# Autodesk Inventor assembly: PCBPT_V3_V2
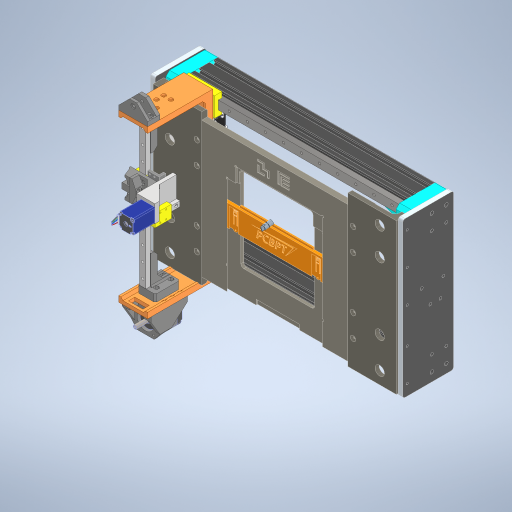
[picture p0: Inventor's stored thumbnail of the model, 512x512]
Saved by Autodesk Inventor 2024.1 (Build 281209000, 209)
## iProperties
Created: 2023-09-27
Part Number: PCBPT_V3_V2
Document SubType Name: Assembly
Designer: l1534
Author: l1534
## Documents named in this file (29)
- C:\DATA\Documents\Lab\github\PCBPT\PCBPT_V3\Mechanical\Mechanical_2\PCBPT_V3_V2.iam
- C:\DATA\Documents\Lab\github\PCBPT\PCBPT_V3\Mechanical\Mechanical_2\Nema 17 Stepper Motor - 40mm - 1.8deg, 61oz-in v1 (2).ipt
- C:\DATA\Documents\Lab\github\PCBPT\PCBPT_V3\Mechanical\Mechanical_2\Part 1 (1).ipt
- C:\DATA\Documents\Lab\github\PCBPT\PCBPT_V3\Mechanical\Mechanical_2\Part 1 (2).ipt
- C:\DATA\Documents\Lab\github\PCBPT\PCBPT_V3\Mechanical\Mechanical_2\Part 1 (3).ipt
- C:\DATA\Documents\Lab\github\PCBPT\PCBPT_V3\Mechanical\Mechanical_2\Part 1 (6).ipt
- C:\DATA\Documents\Lab\github\PCBPT\PCBPT_V3\Mechanical\Mechanical_2\Part 1 (21).ipt
- C:\DATA\Documents\Lab\github\PCBPT\PCBPT_V3\Mechanical\Mechanical_2\Part 1 (22).ipt
- C:\DATA\Documents\Lab\github\PCBPT\PCBPT_V3\Mechanical\Mechanical_2\Part 1 (23).ipt
- C:\DATA\Documents\Lab\github\PCBPT\PCBPT_V3\Mechanical\Mechanical_2\Part Studio 1 - Part 1.ipt
- C:\DATA\Documents\Lab\github\PCBPT\PCBPT_V3\Mechanical\Mechanical_2\wall_conn_2 v8 (2).ipt
- C:\DATA\Documents\Lab\github\PCBPT\PCBPT_V3\Mechanical\Mechanical_2\Wall_connector v11 (2).ipt
- C:\DATA\Documents\Lab\github\PCBPT\PCBPT_V3\Mechanical\Mechanical_2\MGN12H_block.ipt
- C:\DATA\Documents\Lab\github\PCBPT\PCBPT_V3\Mechanical\Mechanical_2\MGN12H_rail.ipt
- C:\DATA\Documents\Lab\github\PCBPT\PCBPT_V3\Mechanical\Mechanical_2\MGN9C_block.ipt
- C:\DATA\Documents\Lab\github\PCBPT\PCBPT_V3\Mechanical\Mechanical_2\MGN9x200mm_rail.ipt
- C:\DATA\Documents\Lab\github\PCBPT\PCBPT_V3\Mechanical\6mm 3v laser diode (1)\6mm 3v laser diode (1).ipt
- C:\DATA\Documents\Lab\github\PCBPT\PCBPT_V3\Mechanical\Part 1 (33)\Part 1 (33).ipt
- C:\DATA\Documents\Lab\github\PCBPT\PCBPT_V3\Mechanical\Mechanical_2\Part 1 (41)\Part 1 (41).ipt
- C:\DATA\Documents\Lab\github\PCBPT\PCBPT_V3\Mechanical\Mechanical_2\Part 1 (83)\Part 1 (83).ipt
- C:\DATA\Documents\Lab\github\PCBPT\PCBPT_V3\Mechanical\Mechanical_2\Part 1 (7)\Part 1 (7).ipt
- C:\DATA\Documents\Lab\github\PCBPT\PCBPT_V3\Mechanical\Mechanical_2\SY20STH30-0604A (2)\SY20STH30-0604A (2).ipt
- C:\DATA\Documents\Lab\github\PCBPT\PCBPT_V3\Mechanical\Mechanical_2\Z_motor_holder.ipt
- C:\DATA\Documents\Lab\github\PCBPT\PCBPT_V3\Mechanical\Mechanical_2\MGN7c_50mm_rail.ipt
- C:\DATA\Documents\Lab\github\PCBPT\PCBPT_V3\Mechanical\Mechanical_2\MGN7C_slider.ipt
- C:\DATA\Documents\Lab\github\PCBPT\PCBPT_V3\Mechanical\Mechanical_2\platform - Part 1\platform - Part 1.ipt
- C:\DATA\Documents\Lab\github\PCBPT\PCBPT_V3\Mechanical\Mechanical_2\PCB_clip - Part 1\PCB_clip - Part 1.ipt
- C:\DATA\Documents\Lab\github\PCBPT\PCBPT_V3\Mechanical\Mechanical_2\platform_holder_L - Part 1\platform_holder_L - Part 1.ipt
- C:\DATA\Documents\Lab\github\PCBPT\PCBPT_V3\Mechanical\Mechanical_2\platform_holder_R - Part 1\platform_holder_R - Part 1.ipt
## Components (36 placed, 28 different names)
1. Nema 17 Stepper Motor - 40mm - 1.8deg, 61oz-in v1 (2):1 — Rigid:11
2. Part 1 (1):1 — Rigid:14, Rigid:15, Rigid:16, Rigid:17, Rigid:18, Rigid:25
3. Part 1 (2):1 — Rigid:9, Rigid:11
4. Part 1 (23):1 — Rigid:6, Rigid:7, Mate:6
5. Part Studio 1 - Part 1:1 — Rigid:3, Rigid:4, Rigid:8, Rigid:30
6. wall_conn_2 v8 (2):1 — Rigid:4, Mate:4, Flush:1
7. Wall_connector v11 (2):1 — Rigid:3, Rigid:7, Mate:5
8. Nema 17 Stepper Motor - 40mm - 1.8deg, 61oz-in v1 (2):2 — Rigid:10
9. Part 1 (2):2 — Rigid:8, Rigid:10
10. Part 1 (3):2 — Rigid:16
11. Part 1 (6):2 — Rigid:17, Rigid:20
12. Part 1 (21):2 — Rigid:19
13. Part 1 (22):2 — Rigid:18, Rigid:19
14. Part 1 (23):2 — Rigid:5, Mate:3
15. Part Studio 1 - Part 1:2 — Rigid:1, Rigid:2, Rigid:9, Rigid:29
16. wall_conn_2 v8 (2):2 — Rigid:2, Rigid:6
17. Wall_connector v11 (2):2 — Rigid:1, Rigid:5
18. MGN12H_rail:1 — Mate:2, Mate:3, Mate:4, Flush:1
19. MGN12H_rail:2 — Mate:1, Mate:5, Mate:6
20. MGN12H_block:3 — Rigid:14, Mate:2
21. MGN12H_block:4 — Rigid:15, Mate:1
22. MGN9C_block:1 — Mate:7, Mate:8, Rigid:24
23. MGN9x200mm_rail:1 — Rigid:20, Mate:7, Mate:8
24. 6mm 3v laser diode (1):1
25. Part 1 (33):1 — Rigid:22, Rigid:23, Rigid:24, Rigid:28
26. Part 1 (41):1 — Rigid:22
27. Part 1 (83):1 — Rigid:23
28. Part 1 (7):1 — Rigid:25
29. SY20STH30-0604A (2):1 — Rigid:27
30. Z_motor_holder:1 — Rigid:26, Rigid:27, Rigid:28
31. MGN7c_50mm_rail:1 — Rigid:26, Mate:9, Mate:10
32. MGN7C_slider:1 — Mate:9, Mate:10
33. platform - Part 1:1 — Rigid:31, Mate:11, Mate:12
34. PCB_clip - Part 1:1 — Mate:11, Mate:12
35. platform_holder_L - Part 1:1 — Rigid:29
36. platform_holder_R - Part 1:1 — Rigid:30, Rigid:31
## Relationships (41: WeldJoint 28, Mate 12, Flush 1)
- Rigid:1 [WeldJoint]: Part Studio 1 - Part 1:2 ↔ Wall_connector v11 (2):2
- Rigid:2 [WeldJoint]: Part Studio 1 - Part 1:2 ↔ wall_conn_2 v8 (2):2
- Rigid:3 [WeldJoint]: Part Studio 1 - Part 1:1 ↔ Wall_connector v11 (2):1
- Rigid:4 [WeldJoint]: Part Studio 1 - Part 1:1 ↔ wall_conn_2 v8 (2):1
- Rigid:5 [WeldJoint]: Part 1 (23):2 ↔ Wall_connector v11 (2):2
- Rigid:6 [WeldJoint]: Part 1 (23):1 ↔ wall_conn_2 v8 (2):2
- Rigid:7 [WeldJoint]: Part 1 (23):1 ↔ Wall_connector v11 (2):1
- Rigid:8 [WeldJoint]: Part Studio 1 - Part 1:1 ↔ Part 1 (2):2
- Rigid:9 [WeldJoint]: Part 1 (2):1 ↔ Part Studio 1 - Part 1:2
- Rigid:10 [WeldJoint]: Nema 17 Stepper Motor - 40mm - 1.8deg, 61oz-in v1 (2):2 ↔ Part 1 (2):2
- Rigid:11 [WeldJoint]: Nema 17 Stepper Motor - 40mm - 1.8deg, 61oz-in v1 (2):1 ↔ Part 1 (2):1
- Rigid:14 [WeldJoint]: Part 1 (1):1 ↔ MGN12H_block:3
- Rigid:15 [WeldJoint]: Part 1 (1):1 ↔ MGN12H_block:4
- Rigid:16 [WeldJoint]: Part 1 (1):1 ↔ Part 1 (3):2
- Rigid:17 [WeldJoint]: Part 1 (1):1 ↔ Part 1 (6):2
- Rigid:18 [WeldJoint]: Part 1 (1):1 ↔ Part 1 (22):2
- Rigid:19 [WeldJoint]: Part 1 (21):2 ↔ Part 1 (22):2
- Mate:1: MGN12H_rail:2 ↔ MGN12H_block:4
- Mate:2: MGN12H_rail:1 ↔ MGN12H_block:3
- Mate:3: Part 1 (23):2 ↔ MGN12H_rail:1
- Mate:4: wall_conn_2 v8 (2):1 ↔ MGN12H_rail:1
- Flush:1 (4 mm): wall_conn_2 v8 (2):1 ↔ MGN12H_rail:1
- Mate:5: Wall_connector v11 (2):1 ↔ MGN12H_rail:2
- Mate:6: Part 1 (23):1 ↔ MGN12H_rail:2
- Rigid:20 [WeldJoint]: Part 1 (6):2 ↔ MGN9x200mm_rail:1
- Mate:7: MGN9C_block:1 ↔ MGN9x200mm_rail:1
- Mate:8: MGN9C_block:1 ↔ MGN9x200mm_rail:1
- Rigid:22 [WeldJoint]: Part 1 (33):1 ↔ Part 1 (41):1
- Rigid:23 [WeldJoint]: Part 1 (33):1 ↔ Part 1 (83):1
- Rigid:24 [WeldJoint]: MGN9C_block:1 ↔ Part 1 (33):1
- Rigid:25 [WeldJoint]: Part 1 (1):1 ↔ Part 1 (7):1
- Rigid:26 [WeldJoint]: Z_motor_holder:1 ↔ MGN7c_50mm_rail:1
- Mate:9: MGN7c_50mm_rail:1 ↔ MGN7C_slider:1
- Mate:10: MGN7c_50mm_rail:1 ↔ MGN7C_slider:1
- Rigid:27 [WeldJoint]: SY20STH30-0604A (2):1 ↔ Z_motor_holder:1
- Rigid:28 [WeldJoint]: Part 1 (33):1 ↔ Z_motor_holder:1
- Rigid:29 [WeldJoint]: Part Studio 1 - Part 1:2 ↔ platform_holder_L - Part 1:1
- Rigid:30 [WeldJoint]: Part Studio 1 - Part 1:1 ↔ platform_holder_R - Part 1:1
- Rigid:31 [WeldJoint]: platform - Part 1:1 ↔ platform_holder_R - Part 1:1
- Mate:11: platform - Part 1:1 ↔ PCB_clip - Part 1:1
- Mate:12: platform - Part 1:1 ↔ PCB_clip - Part 1:1
